# Autodesk Inventor assembly: ЛЦМК0000002.00.00.00.00.10
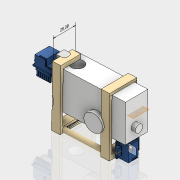
[picture p0: Inventor's stored thumbnail of the model, 180x180]
Saved by Autodesk Inventor 2021.2 (Build 252289000, 289)
## iProperties
Created: 2025-10-23
Part Number: ЛЦМК0000002.00.00.00.00.10
Document SubType Name: Assembly
Designer: Захаров
Author: Захаров
## Documents named in this file (6)
- C:\Users\Public\Documents\Kingroon\Models\CaseARHead1\ЛЦМК0000002.00.00.00.00.10.iam
- C:\Users\Public\Documents\Kingroon\Models\CaseARHead1\ЛЦМК0000002.00.00.00.00.05.ipt
- C:\Users\Public\Documents\Kingroon\Models\CaseARHead1\Сборка1.iam
- C:\Users\Public\Documents\Kingroon\Models\CaseARHead1\ЛЦМК000002.00.00.00.00.06.ipt
- C:\Users\Public\Documents\Kingroon\Models\CaseARHead1\ЛЦМК000002.00.00.00.00.02.ipt
- C:\Users\Public\Documents\Kingroon\Models\CaseARHead1\ЛЦМК000002.00.00.00.00.07.ipt
## Components (6 placed, 5 different names)
1. ЛЦМК0000002.00.00.00.00.05:1 — Совмещение:1, Заподлицо:1, Заподлицо:2, Совмещение:2, Заподлицо:3, Заподлицо:4, Совмещение:3, Совмещение:4, Совмещение:5, Flush:5, Flush:6
2. Сборка1:1 [sub-assembly] — Совмещение:1, Заподлицо:1, Заподлицо:2, Совмещение:6
3. Сборка1:2 [sub-assembly] — Совмещение:2, Заподлицо:3, Заподлицо:4, Flush:7
4. ЛЦМК000002.00.00.00.00.06:1 — Совмещение:6
5. ЛЦМК000002.00.00.00.00.02:1 — Совмещение:3, Совмещение:4, Совмещение:5, Flush:5, Flush:6
6. ЛЦМК000002.00.00.00.00.07:1 — Flush:7
## Relationships (13: Flush 7, Mate 6)
- Совмещение:1 [Mate] (3 mm): ЛЦМК0000002.00.00.00.00.05:1 ↔ Сборка1:1
- Заподлицо:1 [Flush]: ЛЦМК0000002.00.00.00.00.05:1 ↔ Сборка1:1
- Заподлицо:2 [Flush] (2.4 mm): ЛЦМК0000002.00.00.00.00.05:1 ↔ Сборка1:1
- Совмещение:2 [Mate] (3 mm): ЛЦМК0000002.00.00.00.00.05:1 ↔ Сборка1:2
- Заподлицо:3 [Flush] (3 mm): ЛЦМК0000002.00.00.00.00.05:1 ↔ Сборка1:2
- Заподлицо:4 [Flush] (3 mm): ЛЦМК0000002.00.00.00.00.05:1 ↔ Сборка1:2
- Совмещение:3 [Mate]: ЛЦМК0000002.00.00.00.00.05:1 ↔ ЛЦМК000002.00.00.00.00.02:1
- Совмещение:4 [Mate]: ЛЦМК0000002.00.00.00.00.05:1 ↔ ЛЦМК000002.00.00.00.00.02:1
- Совмещение:5 [Mate]: ЛЦМК0000002.00.00.00.00.05:1 ↔ ЛЦМК000002.00.00.00.00.02:1
- Совмещение:6 [Mate]: Сборка1:1 ↔ ЛЦМК000002.00.00.00.00.06:1
- Flush:5: ЛЦМК0000002.00.00.00.00.05:1 ↔ ЛЦМК000002.00.00.00.00.02:1
- Flush:6: ЛЦМК0000002.00.00.00.00.05:1 ↔ ЛЦМК000002.00.00.00.00.02:1
- Flush:7: Сборка1:2 ↔ ЛЦМК000002.00.00.00.00.07:1
